# Autodesk Inventor assembly: four_bar_linkage_v1
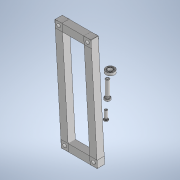
[picture p0: Inventor's stored thumbnail of the model, 180x180]
Saved by Autodesk Inventor 2022 (Build 260153000, 153)
## iProperties
Created: 2022-05-22
Part Number: four_bar_linkage_v1
Document SubType Name: Assembly
Designer: kylem
Author: kylem
## Documents named in this file (6)
- C:\Users\kylem\OneDrive\Documents\GitHub\IMML_Contactile_Gripper_Hardware\gripper_v2\four_bar_linkage_v1.iam
- C:\Users\kylem\OneDrive\Documents\GitHub\IMML_Contactile_Gripper_Hardware\gripper_v2\parallel_bar_long_v1.ipt
- C:\Users\kylem\OneDrive\Documents\GitHub\IMML_Contactile_Gripper_Hardware\gripper_v2\parallel_bar_short_v1.ipt
- C:\Users\kylem\Downloads\95648A270_Captive Pins.ipt
- C:\Users\kylem\Downloads\95648A350_Captive Pins.ipt
- C:\Users\kylem\Downloads\57155K344_Stainless Steel Ball Bearing.ipt
## Components (7 placed, 5 different names)
1. parallel_bar_long_v1:1 — Flush:3, Mate:4, Mate:6
2. parallel_bar_short_v1:1 — Flush:4, Mate:5, Mate:6
3. parallel_bar_long_v1:2 — Mate:3, Flush:2, Flush:4, Mate:5
4. parallel_bar_short_v1:2 — Mate:1, Mate:2, Flush:1, Mate:3, Flush:2, Flush:3, Mate:4
5. 95648A270_Captive Pins:1
6. 95648A350_Captive Pins:1
7. 57155K344_Stainless Steel Ball Bearing:1
## Relationships (10: Mate 6, Flush 4)
- Mate:1: parallel_bar_short_v1:2
- Mate:2: parallel_bar_short_v1:2
- Flush:1: parallel_bar_short_v1:2
- Mate:3: parallel_bar_long_v1:2 ↔ parallel_bar_short_v1:2
- Flush:2: parallel_bar_long_v1:2 ↔ parallel_bar_short_v1:2
- Flush:3: parallel_bar_long_v1:1 ↔ parallel_bar_short_v1:2
- Mate:4: parallel_bar_long_v1:1 ↔ parallel_bar_short_v1:2
- Flush:4: parallel_bar_short_v1:1 ↔ parallel_bar_long_v1:2
- Mate:5: parallel_bar_short_v1:1 ↔ parallel_bar_long_v1:2
- Mate:6: parallel_bar_long_v1:1 ↔ parallel_bar_short_v1:1
